# Autodesk Inventor assembly: bmpAssembly
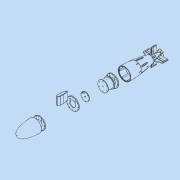
[picture p0: Inventor's stored thumbnail of the model, 180x180]
Saved by Autodesk Inventor 2017 (Build 210142000, 142)
## iProperties
Created: 2016-12-14
Part Number: bmpAssembly
Document SubType Name: Assembly
Designer: techn
Author: techn
## Documents named in this file (13)
- D:\OneDrive\Documents\Other Projects\Submarine\CAD\bmpAssembly.iam
- D:\OneDrive\Documents\Other Projects\Submarine\CAD\midships\PrimaryHullLexanTube_01.ipt
- D:\OneDrive\Documents\Other Projects\Submarine\CAD\fore\primarySingleFore_02.ipt
- D:\OneDrive\Documents\Other Projects\Submarine\CAD\aft\RearmostAftSectionAssembly0.iam
- D:\OneDrive\Documents\Other Projects\Submarine\CAD\aft\AftSectionAirtightRear.ipt
- D:\OneDrive\Documents\Other Projects\Submarine\CAD\aft\AftSectionWithSteeringLinkages.ipt
- D:\OneDrive\Documents\Other Projects\Submarine\CAD\midships\Sail\solidSail.ipt
- D:\OneDrive\Documents\Other Projects\Submarine\CAD\aft\propeller.ipt
- D:\OneDrive\Documents\Other Projects\Submarine\CAD\aft\aftSectionAirtightCap.ipt
- D:\OneDrive\Documents\Other Projects\Submarine\CAD\midships\BallastSection\pistonTank.ipt
- D:\OneDrive\Documents\Other Projects\Submarine\CAD\midships\SpoolSection\Spool.ipt
- D:\OneDrive\Documents\Other Projects\Submarine\CAD\midships\SpoolSection\SpoolEndFrontSide.ipt
- D:\OneDrive\Documents\Other Projects\Submarine\CAD\midships\BallastSection\pistonSealingDisc.ipt
## Components (15 placed, 12 different names)
1. PrimaryHullLexanTube_01:1 — Mate:1, Mate:2, Mate:3, Mate:4, Mate:11, Mate:12, Mate:15, Mate:16, Mate:17, Mate:18, Mate:23
2. primarySingleFore_02:1 — Mate:1, Mate:2
3. RearmostAftSectionAssembly0:1 [sub-assembly] — Mate:7, Mate:8, Angle:1, Mate:9, Mate:13, Mate:14
4. AftSectionWithSteeringLinkages:1 — Mate:5, Mate:6, Mate:7, Mate:8, Mate:9, Mate:10
5. solidSail:1 — Mate:11, Angle:2, Mate:12
6. AftSectionAirtightRear:1 — Mate:3, Mate:4, Mate:5, Mate:6, Mate:10
7. propeller:1 — Mate:13, Mate:14
8. aftSectionAirtightCap:1 — Mate:15
9. aftSectionAirtightCap:2 — Mate:17
10. aftSectionAirtightCap:3 — Mate:16, Mate:24, Mate:25
11. pistonTank:1 — Mate:18, Mate:24
12. Spool:1 — Mate:19, Mate:20, Mate:21, Mate:22, Mate:23
13. SpoolEndFrontSide:1 — Mate:20, Mate:22
14. SpoolEndFrontSide:2 — Mate:19, Mate:21
15. pistonSealingDisc:1 — Mate:25
## Relationships (27: Mate 25, Angle 2)
- Mate:1: PrimaryHullLexanTube_01:1 ↔ primarySingleFore_02:1
- Mate:2: PrimaryHullLexanTube_01:1 ↔ primarySingleFore_02:1
- Mate:3: PrimaryHullLexanTube_01:1 ↔ AftSectionAirtightRear:1
- Mate:4: PrimaryHullLexanTube_01:1 ↔ AftSectionAirtightRear:1
- Mate:5: AftSectionWithSteeringLinkages:1 ↔ AftSectionAirtightRear:1
- Mate:6: AftSectionWithSteeringLinkages:1 ↔ AftSectionAirtightRear:1
- Mate:7: RearmostAftSectionAssembly0:1 ↔ AftSectionWithSteeringLinkages:1
- Mate:8: RearmostAftSectionAssembly0:1 ↔ AftSectionWithSteeringLinkages:1
- Angle:1 (0 deg): RearmostAftSectionAssembly0:1
- Mate:9: RearmostAftSectionAssembly0:1 ↔ AftSectionWithSteeringLinkages:1
- Mate:10: AftSectionWithSteeringLinkages:1 ↔ AftSectionAirtightRear:1
- Mate:11: PrimaryHullLexanTube_01:1 ↔ solidSail:1
- Angle:2 (0 deg): solidSail:1
- Mate:12 (-190.5 mm): PrimaryHullLexanTube_01:1 ↔ solidSail:1
- Mate:13: RearmostAftSectionAssembly0:1 ↔ propeller:1
- Mate:14: RearmostAftSectionAssembly0:1 ↔ propeller:1
- Mate:15: PrimaryHullLexanTube_01:1 ↔ aftSectionAirtightCap:1
- Mate:16: PrimaryHullLexanTube_01:1 ↔ aftSectionAirtightCap:3
- Mate:17: PrimaryHullLexanTube_01:1 ↔ aftSectionAirtightCap:2
- Mate:18: PrimaryHullLexanTube_01:1 ↔ pistonTank:1
- Mate:19: Spool:1 ↔ SpoolEndFrontSide:2
- Mate:20: Spool:1 ↔ SpoolEndFrontSide:1
- Mate:21: Spool:1 ↔ SpoolEndFrontSide:2
- Mate:22: Spool:1 ↔ SpoolEndFrontSide:1
- Mate:23: PrimaryHullLexanTube_01:1 ↔ Spool:1
- Mate:24 (6.35 mm): aftSectionAirtightCap:3 ↔ pistonTank:1
- Mate:25: aftSectionAirtightCap:3 ↔ pistonSealingDisc:1
